# Autodesk Inventor assembly: JWM
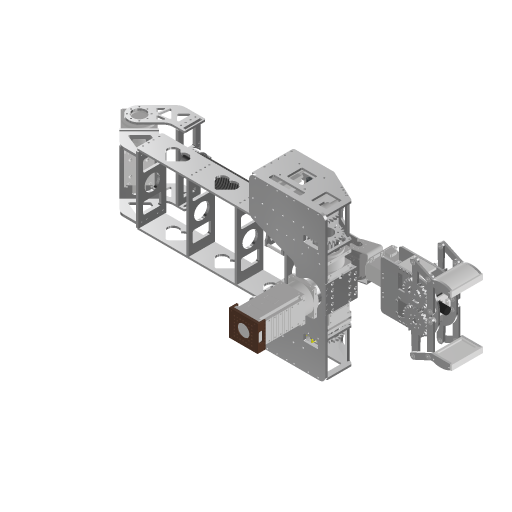
[picture p0: Inventor's stored thumbnail of the model, 512x512]
Saved by Autodesk Inventor 2023.2 (Build 272271000, 271)
## iProperties
Created: 2022-01-18
Part Number: JWM
Document SubType Name: Assembly
Designer: BAEK
Mass: 6819.61 g
Surface Area: 11704.2 cm^2
Volume: 2901.05 cm^3
Density: 2.35074 g/cm^3
Author: BAEK
## iProperties of the stored document 4파이 45.ipt
Created: 2014-03-10
Part Number: 4파이 45
Material: 일반
Description: STEP AP203
Document SubType Name: Modeling
Designer: BAEK
Density: 1 g/cm^3
Appearance: 기본값
Mass: 0.700163 g
Surface Area: 7.4178 cm^2
Volume: 0.700163 cm^3
Sending System: SolidWorks 2007
Preprocessor: SwSTEP 2.0
Title: CSH-STN-M4-45_203.STEP
Author: guan-li
Revision Number: ANY
## iProperties of the stored document 4파이 40.ipt
Created: 2014-03-10
Part Number: 4파이 40
Material: 일반
Description: STEP AP203
Document SubType Name: Modeling
Designer: BAEK
Density: 1 g/cm^3
Appearance: 기본값
Mass: 0.637331 g
Surface Area: 6.78949 cm^2
Volume: 0.637331 cm^3
Sending System: SolidWorks 2007
Preprocessor: SwSTEP 2.0
Title: CSH-STN-M4-40_203.STEP
Author: guan-li
Revision Number: ANY
## Documents named in this file (63)
- C:\Users\BAEK\Desktop\JWM\JWM.iam
- C:\Users\BAEK\Desktop\JWM\매니퓰레이터\큰모터.ipt
- C:\Users\BAEK\Desktop\JWM\매니퓰레이터\큰모터사이드_4T.ipt
- C:\Users\BAEK\Desktop\JWM\매니퓰레이터\큰모터아이들러.ipt
- C:\Users\BAEK\Desktop\JWM\매니퓰레이터\조인트3_힌지아랫판_4T.ipt
- C:\Users\BAEK\Desktop\JWM\매니퓰레이터\조인트3_힌지윗판_4T.ipt
- C:\Users\BAEK\Desktop\JWM\매니퓰레이터\조인트3_힌지사이드_6T.ipt
- C:\Users\BAEK\Desktop\JWM\매니퓰레이터\조인트3힌지사이드_4T.ipt
- C:\Users\BAEK\Desktop\JWM\매니퓰레이터\조인트3힌지윗판_6T.ipt
- C:\Users\BAEK\Desktop\JWM\매니퓰레이터\조인트3링크2연결부.ipt
- C:\Users\BAEK\Desktop\JWM\매니퓰레이터\링크2_200mm.ipt
- C:\Users\BAEK\Desktop\JWM\매니퓰레이터\조인트4링크2연결부.ipt
- C:\Users\BAEK\Desktop\JWM\매니퓰레이터\조인트4박스구조1_4T.ipt
- C:\Users\BAEK\Desktop\JWM\매니퓰레이터\조인트4박스구조2_4T.ipt
- C:\Users\BAEK\Desktop\JWM\매니퓰레이터\MX64.ipt
- C:\Users\BAEK\Desktop\JWM\매니퓰레이터\조인트4플랜지_2T.ipt
- C:\Users\BAEK\Desktop\JWM\매니퓰레이터\MX106.ipt
- C:\Users\BAEK\Desktop\JWM\매니퓰레이터\조인트1베어링관철혼_8T_2pi가공.ipt
- C:\Users\BAEK\Desktop\JWM\매니퓰레이터\회로프레임.ipt
- C:\Users\BAEK\Desktop\JWM\매니퓰레이터\조인트4베어링관절1.ipt
- C:\Users\BAEK\Desktop\JWM\매니퓰레이터\조인트4베어링관절2.ipt
- C:\Users\BAEK\Desktop\JWM\매니퓰레이터\조인트4베어링관절3.ipt
- C:\Users\BAEK\Desktop\JWM\매니퓰레이터\조인트4베어링.ipt
- C:\Users\BAEK\Desktop\JWM\매니퓰레이터\조인트4베어링관절혼.ipt
- **C:\Users\BAEK\Desktop\JWM\JWM.iam*LocalDocs*xAaaaamdaAaaaaaaaAaaaafwn4e*4파이 45.ipt
- C:\Users\BAEK\Desktop\JWM\매니퓰레이터\4파이너트.ipt
- **C:\Users\BAEK\Desktop\JWM\JWM.iam*LocalDocs*xAaaaqwaaAaaaaaaaAaaaazuaFb*4파이 40.ipt
- C:\Users\BAEK\Desktop\JWM\매니퓰레이터\J1J2_Bottom.ipt
- C:\Users\BAEK\Desktop\JWM\매니퓰레이터\J1J2_Side.ipt
- C:\Users\BAEK\Desktop\JWM\매니퓰레이터\J1J2_Top.ipt
- C:\Users\BAEK\Desktop\JWM\매니퓰레이터\J2L1_H_Top.ipt
- C:\Users\BAEK\Desktop\JWM\매니퓰레이터\기어1.ipt
- C:\Users\BAEK\Desktop\JWM\매니퓰레이터\기어2.ipt
- C:\Users\BAEK\Desktop\JWM\매니퓰레이터\6파이베어링.ipt
- C:\Users\BAEK\Desktop\JWM\매니퓰레이터\큰기어 와셔.ipt
- C:\Users\BAEK\Desktop\JWM\매니퓰레이터\너트6.ipt
- C:\Users\BAEK\Desktop\JWM\매니퓰레이터\조인트5힌지사이드1_2T.ipt
- C:\Users\BAEK\Desktop\JWM\매니퓰레이터\조인트5힌지사이드2_2T.ipt
- C:\Users\BAEK\Desktop\JWM\매니퓰레이터\큰기어 와셔2t.ipt
- C:\Users\BAEK\Desktop\JWM\매니퓰레이터\J2L1_H_Side2.ipt
- C:\Users\BAEK\Desktop\JWM\매니퓰레이터\ATHC8-MB_b.ipt
- C:\Users\BAEK\Desktop\JWM\매니퓰레이터\사이드프레임.ipt
- C:\Users\BAEK\Desktop\JWM\매니퓰레이터\C-LHFC8.ipt
- C:\Users\BAEK\Desktop\JWM\매니퓰레이터\스프링블럭2.ipt
- C:\Users\BAEK\Desktop\JWM\매니퓰레이터\FWSSA-D6-V3-T7.ipt
- C:\Users\BAEK\Desktop\JWM\매니퓰레이터\지지프레임1.ipt
- C:\Users\BAEK\Desktop\JWM\매니퓰레이터\지지프레임2.ipt
- C:\Users\BAEK\Desktop\JWM\매니퓰레이터\축지지프레임.ipt
- C:\Users\BAEK\Desktop\JWM\매니퓰레이터\스프링2.ipt
- C:\Users\BAEK\Desktop\JWM\매니퓰레이터\RDOB8-86-WMC4.ipt
- C:\Users\BAEK\Desktop\JWM\매니퓰레이터\RDOB6-86-WMC3.ipt
- C:\Users\BAEK\Desktop\JWM\그리퍼\Assemble.iam
- C:\Users\BAEK\Desktop\JWM\매니퓰레이터\lm가이드가이드.ipt
- C:\Users\BAEK\Desktop\JWM\매니퓰레이터\SSEBZ-MX16_b.ipt
- C:\Users\BAEK\Desktop\JWM\매니퓰레이터\SSEBZ-MX16-70_r.ipt
- C:\Users\BAEK\Desktop\JWM\매니퓰레이터\사이드프레임2.ipt
- C:\Users\BAEK\Desktop\JWM\매니퓰레이터\FRP54-A110.ipt
- C:\Users\BAEK\Desktop\JWM\매니퓰레이터\Supporter30.ipt
- C:\Users\BAEK\Desktop\JWM\매니퓰레이터\ATHC6-MB_b.ipt
- **C:\Users\PARK\Desktop\2022 manipulator (국방로봇)\JWM.iam*LocalDocs*xAaaaamdaAaaaaaaaAaaaafwn4e*4파이 45.ipt
- **C:\Users\PARK\Desktop\2022 manipulator (국방로봇)\JWM.iam*LocalDocs*xAaaaqwaaAaaaaaaaAaaaazuaFb*4파이 40.ipt
- C:\Users\BAEK\Desktop\JWM\매니퓰레이터\4파이 45.STEP
- C:\Users\BAEK\Desktop\JWM\매니퓰레이터\4파이 40.STEP
## Components (139 placed, 58 different names)
1. 큰모터:1 — 삽입:238, 삽입:239, 삽입:1328, 삽입:1329
2. 큰모터:2 — 삽입:725, 삽입:726, 삽입:994, 삽입:995, 삽입:997, 삽입:998, 삽입:1369
3. 조인트3_힌지사이드_6T:3 — 삽입:105, 삽입:1330
4. 조인트3_힌지사이드_6T:4 — 삽입:104, 삽입:1331, 삽입:1347
5. 큰모터:3 — 삽입:96, 삽입:97, 삽입:98, 삽입:99, 삽입:102, 삽입:103, 삽입:1390
6. 큰모터사이드_4T:3 — 삽입:96, 삽입:97, 삽입:101
7. 큰모터사이드_4T:4 — 삽입:98, 삽입:99, 삽입:100
8. 큰모터아이들러:2 — 삽입:100, 삽입:101, 삽입:1387, 삽입:1402
9. 조인트3_힌지윗판_4T:2 — 삽입:102, 삽입:103, 삽입:104, 삽입:105, 삽입:264, 삽입:265
10. 조인트3힌지윗판_6T:1 — 삽입:130, 삽입:131, 삽입:132, 삽입:133, 삽입:1388, 삽입:1389, 삽입:1391
11. 조인트3링크2연결부:1 — 삽입:130, 삽입:131, 플러쉬:3
12. 조인트3링크2연결부:2 — 삽입:132, 삽입:133, 삽입:134
13. 링크2_200mm:1 — 삽입:134, 삽입:147
14. 조인트4링크2연결부:2 — 삽입:137, 삽입:138, 삽입:147, 삽입:163
15. 조인트4링크2연결부:3 — 삽입:137, 삽입:138, 플러쉬:3, 삽입:162
16. 조인트4박스구조2_4T:1 — 삽입:148, 삽입:149, 삽입:644, 삽입:646, 삽입:688, 삽입:689, 삽입:1394, 삽입:1395, 삽입:1396, 삽입:1397
17. MX64:1 — 삽입:148, 삽입:149, 삽입:585, 삽입:586, 삽입:587, 삽입:588
18. 조인트4플랜지_2T:1 — 삽입:262, 삽입:263, 삽입:589, 삽입:590
19. 조인트4박스구조1_4T:2 — 삽입:162, 삽입:163, 삽입:1398, 삽입:1399
20. MX106:1 — 삽입:262, 삽입:263, 삽입:1407, 삽입:1408
21. 조인트1베어링관철혼_8T_2pi가공:1 — 삽입:238, 삽입:239, 삽입:1194, 메이트:112
22. 회로프레임:1 — 삽입:264, 삽입:265
23. 조인트4베어링관절1:1 — 삽입:585, 삽입:586, 삽입:648, 삽입:649
24. 조인트4베어링관절2:1
25. 조인트4베어링관절3:1
26. 조인트4베어링:1
27. 조인트4베어링관절혼:1 — 삽입:587, 삽입:588, 삽입:589, 삽입:590
28. 4파이 45:3 — 삽입:644
29. 4파이 45:5 — 삽입:646
30. 4파이너트:3 — 삽입:648
31. 4파이너트:4 — 삽입:649
32. 4파이 40:1 — 삽입:688
33. 4파이 40:2 — 삽입:689
34. J1J2_Side:1 — 삽입:873, 삽입:874
35. J1J2_Side:2 — 삽입:725, 삽입:726, 삽입:727, 삽입:728, 삽입:1195, 삽입:1196
36. J1J2_Top:1 — 삽입:727, 삽입:728, 삽입:873, 삽입:874
37. J2L1_H_Top:1 — 각도:2
38. 큰모터사이드_4T:5 — 삽입:997, 삽입:998, 삽입:1000
39. 큰모터사이드_4T:6 — 삽입:994, 삽입:995, 삽입:999
40. 큰모터아이들러:13 — 삽입:999, 삽입:1000, 삽입:1147, 삽입:1197, 삽입:1352
41. 큰기어 와셔:10 — 삽입:1372, 삽입:1373
42. 큰기어 와셔:11
43. 기어1:17
44. 너트6:20 — 삽입:1161
45. 기어2:4 — 삽입:1170, 삽입:1275, 삽입:1314
46. 큰모터아이들러:15 — 삽입:1225, 삽입:1226
47. 큰기어 와셔2t:4 — 삽입:1275, 삽입:1314
48. ATHC8-MB_b:4 — 메이트:111, 삽입:1244, 삽입:1245
49. RDOB8-86-WMC4:1 — 메이트:134, 삽입:1376
50. RDOB8-86-WMC4:2 — 메이트:122, 메이트:123, 삽입:1277
51. 스프링블럭2:3 — 삽입:1120, 삽입:1121, 접선:3, 삽입:1295, 삽입:1296
52. C-LHFC8:7 — 삽입:1120
53. C-LHFC8:8 — 삽입:1121
54. FWSSA-D6-V3-T7:2 — 삽입:1197
55. FWSSA-D6-V3-T7:3 — 삽입:1147
56. 너트6:23 — 삽입:1161, 삽입:1164
57. 6파이베어링:27 — 삽입:1204
58. 너트6:24
59. 6파이베어링:29 — 삽입:1164, 삽입:1202
60. 너트6:26 — 삽입:1170
61. 너트6:27
62. 6파이베어링:30 — 삽입:1205, 접선:2
63. 너트6:28
64. 6파이베어링:31 — 삽입:1203
65. 지지프레임1:2 — 삽입:1257, 삽입:1258, 삽입:1313
66. 지지프레임2:2 — 삽입:1312, 삽입:1368
67. RDOB6-86-WMC3:1 — 메이트:120
68. 스프링2:5
69. 스프링2:6 — 메이트:111
70. 스프링2:7 — 메이트:125
71. 사이드프레임:8 — 삽입:1200, 삽입:1201, 삽입:1223, 삽입:1224, 삽입:1257, 삽입:1258
72. 큰기어 와셔:12 — 삽입:1361, 삽입:1362
73. 큰기어 와셔:13
74. 기어1:18
75. 사이드프레임:11 — 삽입:1198, 삽입:1199, 삽입:1225, 삽입:1226, 삽입:1263, 삽입:1264
76. J1J2_Bottom:6 — 삽입:1194, 메이트:112, 삽입:1195, 삽입:1196, 삽입:1198, 삽입:1199, 삽입:1200, 삽입:1201, 삽입:1244, 삽입:1245, 삽입:1248, 삽입:1249, 삽입:1250, 삽입:1251, 삽입:1252, 삽입:1253, 메이트:116, 메이트:117, 메이트:118, 메이트:120, 메이트:123, 메이트:134, 각도:2, 삽입:1367, 각도:3
77. 6파이베어링:32 — 삽입:1203, 삽입:1205
78. 6파이베어링:33 — 삽입:1202, 삽입:1204
79. 너트6:29
80. 기어2:5 — 삽입:1276
81. 큰모터아이들러:16 — 삽입:1223, 삽입:1224
82. 큰기어 와셔2t:5 — 삽입:1276
83. 너트6:30
84. 6파이베어링:34 — 접선:3
85. 너트6:31
86. 6파이베어링:35
87. 너트6:32
88. 너트6:33
89. 6파이베어링:36
90. 너트6:34
91. 6파이베어링:37
92. 6파이베어링:38
93. 6파이베어링:39
94. ATHC6-MB_b:1
95. ATHC8-MB_b:6 — 삽입:1248, 삽입:1249, 메이트:122, 메이트:125
96. ATHC8-MB_b:7 — 삽입:1250, 삽입:1251, 메이트:113, 메이트:131
97. ATHC8-MB_b:8 — 삽입:1252, 삽입:1253, 메이트:115, 메이트:133
98. ATHC6-MB_b:2
99. 지지프레임2:3 — 삽입:1365, 삽입:1366
100. 지지프레임1:3 — 삽입:1263, 삽입:1264
101. RDOB8-86-WMC4:5 — 메이트:113, 메이트:116, 메이트:126, 메이트:130, 삽입:1375
102. RDOB6-86-WMC3:3 — 메이트:117, 메이트:128
103. RDOB8-86-WMC4:7 — 메이트:115, 메이트:118, 메이트:129, 삽입:1280
104. 스프링블럭2:4 — 삽입:1272, 접선:2, 삽입:1293, 삽입:1294
105. C-LHFC8:9 — 삽입:1272
106. C-LHFC8:10 — 메이트:126
107. 스프링2:8 — 메이트:130, 메이트:131
108. 스프링2:9 — 메이트:129, 메이트:133
109. 스프링2:10 — 메이트:128
110. 축지지프레임:8 — 삽입:1277, 삽입:1376
111. 축지지프레임:9 — 삽입:1280, 삽입:1375
112. lm가이드가이드:1 — 삽입:1293, 삽입:1294, 삽입:1297, 삽입:1298, 삽입:1299, 삽입:1300
113. lm가이드가이드:2 — 삽입:1295, 삽입:1296, 삽입:1304, 삽입:1305, 삽입:1306, 삽입:1307
114. SSEBZ-MX16_b:1 — 삽입:1297, 삽입:1298, 메이트:135, 메이트:136
115. SSEBZ-MX16_b:2 — 삽입:1299, 삽입:1300, 메이트:137, 메이트:138
116. SSEBZ-MX16-70_r:1 — 메이트:135, 메이트:136, 삽입:1303
117. SSEBZ-MX16-70_r:2 — 메이트:137, 메이트:138, 삽입:1301, 삽입:1302
118. 사이드프레임2:2 — 삽입:1301, 삽입:1302, 삽입:1303, 삽입:1365, 삽입:1366
119. SSEBZ-MX16-70_r:3 — 삽입:1310, 삽입:1311
120. SSEBZ-MX16-70_r:4 — 삽입:1308, 삽입:1309
121. SSEBZ-MX16_b:4 — 삽입:1306, 삽입:1307
122. SSEBZ-MX16_b:5 — 삽입:1304, 삽입:1305
123. 사이드프레임2:3 — 삽입:1308, 삽입:1309, 삽입:1310, 삽입:1311, 삽입:1312, 삽입:1313, 삽입:1367, 삽입:1368
124. FRP54-A110:3 — 삽입:1328, 삽입:1329
125. 조인트3_힌지아랫판_4T:2 — 삽입:1330, 삽입:1331, 삽입:1347, 삽입:1356, 삽입:1357
126. J2L1_H_Top:2 — 삽입:1360, 삽입:1371
127. J2L1_H_Top:4 — 삽입:1354, 삽입:1370, 삽입:1374
128. J2L1_H_Side2:8 — 삽입:1352, 삽입:1354, 삽입:1356, 삽입:1357, 삽입:1360, 삽입:1361, 삽입:1362
129. J2L1_H_Side2:9 — 삽입:1369, 삽입:1370, 삽입:1371, 각도:3, 삽입:1372, 삽입:1373, 삽입:1374
130. 조인트3힌지사이드_4T:6 — 삽입:1387, 삽입:1388, 삽입:1389, 삽입:1402
131. 조인트3힌지사이드_4T:7 — 삽입:1390, 삽입:1391
132. Supporter30:1 — 삽입:1396
133. Supporter30:2 — 삽입:1394, 삽입:1398
134. Supporter30:3 — 삽입:1395, 삽입:1399
135. Supporter30:4 — 삽입:1397
136. 조인트5힌지사이드1_2T:7
137. 조인트5힌지사이드2_2T:7 — 삽입:1407, 삽입:1408
138. MX64:11 — 삽입:1409, 삽입:1410
139. Assemble:13 [sub-assembly] — 삽입:1409, 삽입:1410
## Relationships (239: Insert 198, Mate 36, Tangent 2, Angle 2, Flush 1)
- 삽입:96 [Insert]: 큰모터:3 ↔ 큰모터사이드_4T:3
- 삽입:97 [Insert]: 큰모터:3 ↔ 큰모터사이드_4T:3
- 삽입:98 [Insert]: 큰모터:3 ↔ 큰모터사이드_4T:4
- 삽입:99 [Insert]: 큰모터:3 ↔ 큰모터사이드_4T:4
- 삽입:100 [Insert]: 큰모터사이드_4T:4 ↔ 큰모터아이들러:2
- 삽입:101 [Insert]: 큰모터사이드_4T:3 ↔ 큰모터아이들러:2
- 삽입:102 [Insert]: 큰모터:3 ↔ 조인트3_힌지윗판_4T:2
- 삽입:103 [Insert]: 큰모터:3 ↔ 조인트3_힌지윗판_4T:2
- 삽입:104 [Insert]: 조인트3_힌지사이드_6T:4 ↔ 조인트3_힌지윗판_4T:2
- 삽입:105 [Insert]: 조인트3_힌지사이드_6T:3 ↔ 조인트3_힌지윗판_4T:2
- 삽입:130 [Insert]: 조인트3힌지윗판_6T:1 ↔ 조인트3링크2연결부:1
- 삽입:131 [Insert]: 조인트3힌지윗판_6T:1 ↔ 조인트3링크2연결부:1
- 삽입:132 [Insert]: 조인트3힌지윗판_6T:1 ↔ 조인트3링크2연결부:2
- 삽입:133 [Insert]: 조인트3힌지윗판_6T:1 ↔ 조인트3링크2연결부:2
- 삽입:134 [Insert]: 조인트3링크2연결부:2 ↔ 링크2_200mm:1
- 삽입:137 [Insert]: 조인트4링크2연결부:2 ↔ 조인트4링크2연결부:3
- 삽입:138 [Insert]: 조인트4링크2연결부:2 ↔ 조인트4링크2연결부:3
- 삽입:147 [Insert]: 링크2_200mm:1 ↔ 조인트4링크2연결부:2
- 플러쉬:3 [Flush]: 조인트3링크2연결부:1 ↔ 조인트4링크2연결부:3
- 삽입:148 [Insert]: 조인트4박스구조2_4T:1 ↔ MX64:1
- 삽입:149 [Insert]: 조인트4박스구조2_4T:1 ↔ MX64:1
- 삽입:162 [Insert]: 조인트4링크2연결부:3 ↔ 조인트4박스구조1_4T:2
- 삽입:163 [Insert]: 조인트4링크2연결부:2 ↔ 조인트4박스구조1_4T:2
- 삽입:238 [Insert]: 큰모터:1 ↔ 조인트1베어링관철혼_8T_2pi가공:1
- 삽입:239 [Insert]: 큰모터:1 ↔ 조인트1베어링관철혼_8T_2pi가공:1
- 삽입:262 [Insert]: 조인트4플랜지_2T:1 ↔ MX106:1
- 삽입:263 [Insert]: 조인트4플랜지_2T:1 ↔ MX106:1
- 삽입:264 [Insert]: 조인트3_힌지윗판_4T:2 ↔ 회로프레임:1
- 삽입:265 [Insert]: 조인트3_힌지윗판_4T:2 ↔ 회로프레임:1
- [Insert]: 조인트4베어링관절1:1 ↔ 조인트4베어링관절2:1
- [Insert]: 조인트4베어링관절1:1 ↔ 조인트4베어링관절2:1
- [Mate]: 조인트4베어링관절3:1 ↔ 조인트4베어링:1
- [Mate]: 조인트4베어링관절3:1 ↔ 조인트4베어링:1
- [Insert]: 조인트4베어링관절2:1 ↔ 조인트4베어링관절3:1
- [Insert]: 조인트4베어링관절2:1 ↔ 조인트4베어링관절3:1
- 삽입:585 [Insert]: MX64:1 ↔ 조인트4베어링관절1:1
- 삽입:586 [Insert]: MX64:1 ↔ 조인트4베어링관절1:1
- 삽입:587 [Insert]: MX64:1 ↔ 조인트4베어링관절혼:1
- 삽입:588 [Insert]: MX64:1 ↔ 조인트4베어링관절혼:1
- 삽입:589 [Insert]: 조인트4플랜지_2T:1 ↔ 조인트4베어링관절혼:1
- 삽입:590 [Insert]: 조인트4플랜지_2T:1 ↔ 조인트4베어링관절혼:1
- 삽입:644 [Insert]: 조인트4박스구조2_4T:1 ↔ 4파이 45:3
- 삽입:646 [Insert]: 조인트4박스구조2_4T:1 ↔ 4파이 45:5
- 삽입:648 [Insert]: 조인트4베어링관절1:1 ↔ 4파이너트:3
- 삽입:649 [Insert]: 조인트4베어링관절1:1 ↔ 4파이너트:4
- 삽입:688 [Insert]: 조인트4박스구조2_4T:1 ↔ 4파이 40:1
- 삽입:689 [Insert]: 조인트4박스구조2_4T:1 ↔ 4파이 40:2
- 삽입:725 [Insert]: 큰모터:2 ↔ J1J2_Side:2
- 삽입:726 [Insert]: 큰모터:2 ↔ J1J2_Side:2
- 삽입:727 [Insert]: J1J2_Side:2 ↔ J1J2_Top:1
- 삽입:728 [Insert]: J1J2_Side:2 ↔ J1J2_Top:1
- 삽입:873 [Insert]: J1J2_Side:1 ↔ J1J2_Top:1
- 삽입:874 [Insert]: J1J2_Side:1 ↔ J1J2_Top:1
- 삽입:994 [Insert]: 큰모터:2 ↔ 큰모터사이드_4T:6
- 삽입:995 [Insert]: 큰모터:2 ↔ 큰모터사이드_4T:6
- 삽입:997 [Insert]: 큰모터:2 ↔ 큰모터사이드_4T:5
- 삽입:998 [Insert]: 큰모터:2 ↔ 큰모터사이드_4T:5
- 삽입:999 [Insert]: 큰모터사이드_4T:6 ↔ 큰모터아이들러:13
- 삽입:1000 [Insert]: 큰모터사이드_4T:5 ↔ 큰모터아이들러:13
- [Insert]: 큰기어 와셔:10 ↔ 큰기어 와셔:11
- [Insert]: 큰기어 와셔:10 ↔ 큰기어 와셔:11
- [Insert]: 큰기어 와셔:11 ↔ 기어1:17
- [Insert]: 큰기어 와셔:11 ↔ 기어1:17
- [Insert]: 너트6:20 ↔ 기어2:4
- [Insert]: 큰모터아이들러:15 ↔ 큰기어 와셔2t:4
- [Insert]: 큰모터아이들러:15 ↔ 큰기어 와셔2t:4
- [Insert]: 기어2:4 ↔ 큰기어 와셔2t:4
- [Mate]: ATHC8-MB_b:4 ↔ RDOB8-86-WMC4:1
- [Mate]: RDOB8-86-WMC4:2 ↔ 스프링블럭2:3
- [Mate]: RDOB8-86-WMC4:1 ↔ 스프링블럭2:3
- [Mate]: RDOB8-86-WMC4:2 ↔ C-LHFC8:7
- 삽입:1120 [Insert]: 스프링블럭2:3 ↔ C-LHFC8:7
- [Mate]: RDOB8-86-WMC4:1 ↔ C-LHFC8:8
- 삽입:1121 [Insert]: 스프링블럭2:3 ↔ C-LHFC8:8
- 삽입:1147 [Insert]: 큰모터아이들러:13 ↔ FWSSA-D6-V3-T7:3
- [Insert]: 6파이베어링:27 ↔ 너트6:24
- 삽입:1161 [Insert]: 너트6:20 ↔ 너트6:23
- 삽입:1164 [Insert]: 너트6:23 ↔ 6파이베어링:29
- [Insert]: 6파이베어링:30 ↔ 너트6:28
- [Insert]: 너트6:26 ↔ 너트6:27
- [Insert]: 너트6:27 ↔ 6파이베어링:31
- 삽입:1170 [Insert]: 기어2:4 ↔ 너트6:26
- [Mate]: RDOB8-86-WMC4:2 ↔ 스프링2:7
- [Mate]: RDOB6-86-WMC3:1 ↔ 스프링2:5
- [Mate]: RDOB8-86-WMC4:1 ↔ 스프링2:6
- 메이트:111 [Mate]: ATHC8-MB_b:4 ↔ 스프링2:6
- [Insert]: 큰기어 와셔:12 ↔ 큰기어 와셔:13
- [Insert]: 큰기어 와셔:12 ↔ 큰기어 와셔:13
- [Insert]: 큰기어 와셔:13 ↔ 기어1:18
- [Insert]: 큰기어 와셔:13 ↔ 기어1:18
- 삽입:1194 [Insert]: 조인트1베어링관철혼_8T_2pi가공:1 ↔ J1J2_Bottom:6
- 메이트:112 [Mate]: 조인트1베어링관철혼_8T_2pi가공:1 ↔ J1J2_Bottom:6
- 삽입:1195 [Insert]: J1J2_Side:2 ↔ J1J2_Bottom:6
- 삽입:1196 [Insert]: J1J2_Side:2 ↔ J1J2_Bottom:6
- 삽입:1197 [Insert]: 큰모터아이들러:13 ↔ FWSSA-D6-V3-T7:2
- 삽입:1198 [Insert]: 사이드프레임:11 ↔ J1J2_Bottom:6
- 삽입:1199 [Insert]: 사이드프레임:11 ↔ J1J2_Bottom:6
- 삽입:1200 [Insert]: 사이드프레임:8 ↔ J1J2_Bottom:6
- 삽입:1201 [Insert]: 사이드프레임:8 ↔ J1J2_Bottom:6
- 삽입:1202 [Insert]: 6파이베어링:29 ↔ 6파이베어링:33
- 삽입:1203 [Insert]: 6파이베어링:31 ↔ 6파이베어링:32
- 삽입:1204 [Insert]: 6파이베어링:27 ↔ 6파이베어링:33
- 삽입:1205 [Insert]: 6파이베어링:30 ↔ 6파이베어링:32
- [Insert]: 너트6:29 ↔ 기어2:5
- [Insert]: 큰모터아이들러:16 ↔ 큰기어 와셔2t:5
- [Insert]: 큰모터아이들러:16 ↔ 큰기어 와셔2t:5
- [Insert]: 기어2:5 ↔ 큰기어 와셔2t:5
- [Insert]: 6파이베어링:34 ↔ 너트6:31
- [Insert]: 너트6:29 ↔ 너트6:30
- [Insert]: 너트6:30 ↔ 6파이베어링:35
- [Insert]: 6파이베어링:36 ↔ 너트6:34
- [Insert]: 너트6:32 ↔ 너트6:33
- [Insert]: 너트6:33 ↔ 6파이베어링:37
- [Insert]: 기어2:5 ↔ 너트6:32
- [Insert]: 6파이베어링:35 ↔ 6파이베어링:39
- [Insert]: 6파이베어링:37 ↔ 6파이베어링:38
- [Insert]: 6파이베어링:34 ↔ 6파이베어링:39
- [Insert]: 6파이베어링:36 ↔ 6파이베어링:38
- 삽입:1223 [Insert]: 사이드프레임:8 ↔ 큰모터아이들러:16
- 삽입:1224 [Insert]: 사이드프레임:8 ↔ 큰모터아이들러:16
- 삽입:1225 [Insert]: 큰모터아이들러:15 ↔ 사이드프레임:11
- 삽입:1226 [Insert]: 큰모터아이들러:15 ↔ 사이드프레임:11
- 삽입:1244 [Insert]: ATHC8-MB_b:4 ↔ J1J2_Bottom:6
- 삽입:1245 [Insert]: ATHC8-MB_b:4 ↔ J1J2_Bottom:6
- [Insert]: J1J2_Bottom:6 ↔ ATHC6-MB_b:1
- [Insert]: J1J2_Bottom:6 ↔ ATHC6-MB_b:1
- 삽입:1248 [Insert]: J1J2_Bottom:6 ↔ ATHC8-MB_b:6
- 삽입:1249 [Insert]: J1J2_Bottom:6 ↔ ATHC8-MB_b:6
- 삽입:1250 [Insert]: J1J2_Bottom:6 ↔ ATHC8-MB_b:7
- 삽입:1251 [Insert]: J1J2_Bottom:6 ↔ ATHC8-MB_b:7
- 삽입:1252 [Insert]: J1J2_Bottom:6 ↔ ATHC8-MB_b:8
- 삽입:1253 [Insert]: J1J2_Bottom:6 ↔ ATHC8-MB_b:8
- [Insert]: J1J2_Bottom:6 ↔ ATHC6-MB_b:2
- [Insert]: J1J2_Bottom:6 ↔ ATHC6-MB_b:2
- 삽입:1257 [Insert]: 지지프레임1:2 ↔ 사이드프레임:8
- 삽입:1258 [Insert]: 지지프레임1:2 ↔ 사이드프레임:8
- 삽입:1263 [Insert]: 사이드프레임:11 ↔ 지지프레임1:3
- 삽입:1264 [Insert]: 사이드프레임:11 ↔ 지지프레임1:3
- 메이트:113 [Mate]: ATHC8-MB_b:7 ↔ RDOB8-86-WMC4:5
- [Mate]: ATHC6-MB_b:2 ↔ RDOB6-86-WMC3:3
- 메이트:115 [Mate]: ATHC8-MB_b:8 ↔ RDOB8-86-WMC4:7
- 메이트:116 [Mate]: J1J2_Bottom:6 ↔ RDOB8-86-WMC4:5
- 메이트:117 [Mate]: J1J2_Bottom:6 ↔ RDOB6-86-WMC3:3
- 메이트:118 [Mate]: J1J2_Bottom:6 ↔ RDOB8-86-WMC4:7
- [Mate]: RDOB6-86-WMC3:1 ↔ ATHC6-MB_b:1
- 메이트:120 [Mate]: RDOB6-86-WMC3:1 ↔ J1J2_Bottom:6
- [Insert]: 스프링블럭2:4 ↔ C-LHFC8:9
- [Insert]: 스프링블럭2:4 ↔ C-LHFC8:10
- 메이트:122 [Mate]: RDOB8-86-WMC4:2 ↔ ATHC8-MB_b:6
- 메이트:123 [Mate]: RDOB8-86-WMC4:2 ↔ J1J2_Bottom:6
- [Mate]: 스프링2:5 ↔ ATHC6-MB_b:1
- 메이트:125 [Mate]: 스프링2:7 ↔ ATHC8-MB_b:6
- 메이트:126 [Mate]: RDOB8-86-WMC4:5 ↔ C-LHFC8:10
- 삽입:1272 [Insert]: 스프링블럭2:4 ↔ C-LHFC8:9
- 메이트:128 [Mate]: RDOB6-86-WMC3:3 ↔ 스프링2:10
- 메이트:129 [Mate]: RDOB8-86-WMC4:7 ↔ 스프링2:9
- 메이트:130 [Mate]: RDOB8-86-WMC4:5 ↔ 스프링2:8
- 메이트:131 [Mate]: ATHC8-MB_b:7 ↔ 스프링2:8
- [Mate]: ATHC6-MB_b:2 ↔ 스프링2:10
- 메이트:133 [Mate]: ATHC8-MB_b:8 ↔ 스프링2:9
- 접선:2 [Tangent]: 6파이베어링:30 ↔ 스프링블럭2:4
- 메이트:134 [Mate]: RDOB8-86-WMC4:1 ↔ J1J2_Bottom:6
- 삽입:1275 [Insert]: 기어2:4 ↔ 큰기어 와셔2t:4
- 접선:3 [Tangent]: 스프링블럭2:3 ↔ 6파이베어링:34
- 삽입:1276 [Insert]: 기어2:5 ↔ 큰기어 와셔2t:5
- 삽입:1277 [Insert]: RDOB8-86-WMC4:2 ↔ 축지지프레임:8
- 삽입:1280 [Insert]: RDOB8-86-WMC4:7 ↔ 축지지프레임:9
- 각도:2 [Angle] (180 deg): J2L1_H_Top:1 ↔ J1J2_Bottom:6
- 삽입:1293 [Insert]: 스프링블럭2:4 ↔ lm가이드가이드:1
- 삽입:1294 [Insert]: 스프링블럭2:4 ↔ lm가이드가이드:1
- 삽입:1295 [Insert]: 스프링블럭2:3 ↔ lm가이드가이드:2
- 삽입:1296 [Insert]: 스프링블럭2:3 ↔ lm가이드가이드:2
- 삽입:1297 [Insert]: lm가이드가이드:1 ↔ SSEBZ-MX16_b:1
- 삽입:1298 [Insert]: lm가이드가이드:1 ↔ SSEBZ-MX16_b:1
- 삽입:1299 [Insert]: lm가이드가이드:1 ↔ SSEBZ-MX16_b:2
- 삽입:1300 [Insert]: lm가이드가이드:1 ↔ SSEBZ-MX16_b:2
- 메이트:135 [Mate]: SSEBZ-MX16_b:1 ↔ SSEBZ-MX16-70_r:1
- 메이트:136 [Mate]: SSEBZ-MX16_b:1 ↔ SSEBZ-MX16-70_r:1
- 메이트:137 [Mate]: SSEBZ-MX16_b:2 ↔ SSEBZ-MX16-70_r:2
- 메이트:138 [Mate]: SSEBZ-MX16_b:2 ↔ SSEBZ-MX16-70_r:2
- 삽입:1301 [Insert]: SSEBZ-MX16-70_r:2 ↔ 사이드프레임2:2
- 삽입:1302 [Insert]: SSEBZ-MX16-70_r:2 ↔ 사이드프레임2:2
- 삽입:1303 [Insert]: SSEBZ-MX16-70_r:1 ↔ 사이드프레임2:2
- 삽입:1304 [Insert]: lm가이드가이드:2 ↔ SSEBZ-MX16_b:5
- 삽입:1305 [Insert]: lm가이드가이드:2 ↔ SSEBZ-MX16_b:5
- 삽입:1306 [Insert]: lm가이드가이드:2 ↔ SSEBZ-MX16_b:4
- 삽입:1307 [Insert]: lm가이드가이드:2 ↔ SSEBZ-MX16_b:4
- 삽입:1308 [Insert]: SSEBZ-MX16-70_r:4 ↔ 사이드프레임2:3
- 삽입:1309 [Insert]: SSEBZ-MX16-70_r:4 ↔ 사이드프레임2:3
- 삽입:1310 [Insert]: SSEBZ-MX16-70_r:3 ↔ 사이드프레임2:3
- 삽입:1311 [Insert]: SSEBZ-MX16-70_r:3 ↔ 사이드프레임2:3
- 삽입:1312 [Insert]: 지지프레임2:2 ↔ 사이드프레임2:3
- 삽입:1313 [Insert]: 지지프레임1:2 ↔ 사이드프레임2:3
- 삽입:1314 [Insert]: 기어2:4 ↔ 큰기어 와셔2t:4
- 삽입:1328 [Insert]: 큰모터:1 ↔ FRP54-A110:3
- 삽입:1329 [Insert]: 큰모터:1 ↔ FRP54-A110:3
- 삽입:1330 [Insert]: 조인트3_힌지사이드_6T:3 ↔ 조인트3_힌지아랫판_4T:2
- 삽입:1331 [Insert]: 조인트3_힌지사이드_6T:4 ↔ 조인트3_힌지아랫판_4T:2
- 삽입:1347 [Insert]: 조인트3_힌지사이드_6T:4 ↔ 조인트3_힌지아랫판_4T:2
- 삽입:1352 [Insert] (0.5 mm): 큰모터아이들러:13 ↔ J2L1_H_Side2:8
- 삽입:1354 [Insert]: J2L1_H_Top:4 ↔ J2L1_H_Side2:8
- 삽입:1356 [Insert]: 조인트3_힌지아랫판_4T:2 ↔ J2L1_H_Side2:8
- 삽입:1357 [Insert]: 조인트3_힌지아랫판_4T:2 ↔ J2L1_H_Side2:8
- 삽입:1360 [Insert]: J2L1_H_Top:2 ↔ J2L1_H_Side2:8
- 삽입:1361 [Insert]: 큰기어 와셔:12 ↔ J2L1_H_Side2:8
- 삽입:1362 [Insert]: 큰기어 와셔:12 ↔ J2L1_H_Side2:8
- 삽입:1365 [Insert]: 지지프레임2:3 ↔ 사이드프레임2:2
- 삽입:1366 [Insert]: 지지프레임2:3 ↔ 사이드프레임2:2
- 삽입:1367 [Insert]: J1J2_Bottom:6 ↔ 사이드프레임2:3
- 삽입:1368 [Insert]: 지지프레임2:2 ↔ 사이드프레임2:3
- 삽입:1369 [Insert] (0.5 mm): 큰모터:2 ↔ J2L1_H_Side2:9
- 삽입:1370 [Insert]: J2L1_H_Top:4 ↔ J2L1_H_Side2:9
- 삽입:1371 [Insert]: J2L1_H_Top:2 ↔ J2L1_H_Side2:9
- 각도:3 [Angle] (180 deg): J1J2_Bottom:6 ↔ J2L1_H_Side2:9
- 삽입:1372 [Insert]: 큰기어 와셔:10 ↔ J2L1_H_Side2:9
- 삽입:1373 [Insert]: 큰기어 와셔:10 ↔ J2L1_H_Side2:9
- 삽입:1374 [Insert]: J2L1_H_Top:4 ↔ J2L1_H_Side2:9
- 삽입:1375 [Insert]: RDOB8-86-WMC4:5 ↔ 축지지프레임:9
- 삽입:1376 [Insert]: RDOB8-86-WMC4:1 ↔ 축지지프레임:8
- 삽입:1387 [Insert]: 큰모터아이들러:2 ↔ 조인트3힌지사이드_4T:6
- 삽입:1388 [Insert]: 조인트3힌지윗판_6T:1 ↔ 조인트3힌지사이드_4T:6
- 삽입:1389 [Insert]: 조인트3힌지윗판_6T:1 ↔ 조인트3힌지사이드_4T:6
- 삽입:1390 [Insert]: 큰모터:3 ↔ 조인트3힌지사이드_4T:7
- 삽입:1391 [Insert]: 조인트3힌지윗판_6T:1 ↔ 조인트3힌지사이드_4T:7
- 삽입:1394 [Insert]: 조인트4박스구조2_4T:1 ↔ Supporter30:2
- 삽입:1395 [Insert]: 조인트4박스구조2_4T:1 ↔ Supporter30:3
- 삽입:1396 [Insert]: 조인트4박스구조2_4T:1 ↔ Supporter30:1
- 삽입:1397 [Insert]: 조인트4박스구조2_4T:1 ↔ Supporter30:4
- 삽입:1398 [Insert]: 조인트4박스구조1_4T:2 ↔ Supporter30:2
- 삽입:1399 [Insert]: 조인트4박스구조1_4T:2 ↔ Supporter30:3
- 삽입:1402 [Insert]: 큰모터아이들러:2 ↔ 조인트3힌지사이드_4T:6
- [Insert]: 조인트5힌지사이드1_2T:7 ↔ MX64:11
- [Insert]: 조인트5힌지사이드2_2T:7 ↔ MX64:11
- [Insert]: 조인트5힌지사이드1_2T:7 ↔ MX64:11
- [Insert]: 조인트5힌지사이드2_2T:7 ↔ MX64:11
- 삽입:1407 [Insert]: MX106:1 ↔ 조인트5힌지사이드2_2T:7
- 삽입:1408 [Insert]: MX106:1 ↔ 조인트5힌지사이드2_2T:7
- 삽입:1409 [Insert]: MX64:11 ↔ Assemble:13
- 삽입:1410 [Insert]: MX64:11 ↔ Assemble:13
## Named parameters: d1728_d1710 = 0 mm, d1729_d1711 = 0 mm, d1730_d1693 = 0 mm, d1731_d1694 = 0 mm, d1749_d1700 = 0 mm, d1750_d1701 = 0 mm, d1751_d1702 = 0 mm, d1753_d1596_d1515_d1452 = 0 mm, d1862_d1860 = 0 mm, d1869_d1862_d1860 = 0 mm, d1870_d1864 = 0 mm, d1873_d1868 = 0 mm, d1935_d1710 = 0 mm, d1936_d1711 = 0 mm, d1937_d1693 = 0 mm, d1938_d1694 = 0 mm, d1957_d1749_d1700 = 0 mm, d1958_d1750_d1701 = 0 mm, d1959_d1751_d1702 = 0 mm, d1960_d1753_d1596_d1515_d1452 = 0 mm, d1961_d1956 = 0 mm, d1962_d1953 = 0 mm, d1963_d1954 = 0 mm, d1964_d1955 = 0 mm, d1965_d1862_d1860 = 0 mm, d1966_d1864 = 0 mm, d1967_d1868 = 0 mm, d1968_d1869_d1862_d1860 = 0 mm, d1969_d1870_d1864 = 0 mm, d1970_d1873_d1868 = 0 mm, d1971_d1874 = 0 mm, d2032_d1816 = 0 mm, d2033_d1818 = 0 mm, d2237_d2201_d2130_d2079_d1714_d1615_d1506 = 0 mm, d2238_d2202_d2131_d2080_d1715_d1616_d1510 = 0 mm, d2239_d2203_d2132_d2081_d1716_d1618 = 0 mm, d2240_d2204_d2133_d2125 = 0 mm
